# Autodesk Inventor assembly: Drive V3
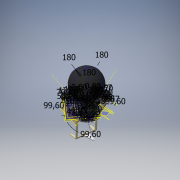
[picture p0: Inventor's stored thumbnail of the model, 180x180]
Saved by Autodesk Inventor 2019.1 (Build 231200000, 200)
## iProperties
Created: 2018-06-30
Part Number: Drive V3
Material: Generisch
Document SubType Name: Assembly
Designer: JochenAlt
Author: JochenAlt
## Documents named in this file (4)
- D:\Projects\Ondine\CAD\Drive V3.iam
- D:\Projects\Ondine\CAD\Sphere.ipt
- D:\Projects\Ondine\CAD\DriveChain V3.iam
- D:\Projects\Ondine\CAD\PCB\ControllerPCBHolder.ipt
## Components (5 placed, 3 different names)
1. Sphere:1 — Passend:38
2. DriveChain V3:1 [sub-assembly] — Passend:39, Passend:40, Passend:41, Passend:42, Passend:43, Passend:45
3. DriveChain V3:2 [sub-assembly] — Passend:39, Passend:40, Passend:41, Passend:42, Passend:44
4. DriveChain V3:3 [sub-assembly] — Passend:44, Passend:45
5. PCBHolder:1
## Relationships (8: Mate 8)
- Passend:38 [Mate]: Sphere:1
- Passend:39 [Mate]: DriveChain V3:1 ↔ DriveChain V3:2
- Passend:40 [Mate]: DriveChain V3:1 ↔ DriveChain V3:2
- Passend:41 [Mate]: DriveChain V3:1 ↔ DriveChain V3:2
- Passend:42 [Mate]: DriveChain V3:1 ↔ DriveChain V3:2
- Passend:43 [Mate]: DriveChain V3:1
- Passend:44 [Mate]: DriveChain V3:2 ↔ DriveChain V3:3
- Passend:45 [Mate]: DriveChain V3:1 ↔ DriveChain V3:3
